# Autodesk Inventor assembly: 110202 DT-20-L1260ZZ
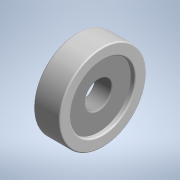
[picture p0: Inventor's stored thumbnail of the model, 180x180]
Saved by Autodesk Inventor 2022.3 (Build 263350000, 350)
## iProperties
Category: PARTsolutions
Company: TOKBEARING
Part Number: 110202 DT-20-L1260ZZ
Catalog Web Link: www.cadenas.de
Description: DT-
Vendor: TOKBEARING
Document SubType Name: Assembly
Designer: partserver
Manufacturer: TOKBEARING
Mass: 1.42292 g
Surface Area: 16.3578 cm^2
Volume: 1.42292 cm^3
Density: 1 g/cm^3
PSOL_IDENT_0: {$CADENAS_DATA\23d-libs\tok_bearing\i_series_bearings\dt_asmtab.prj},192 {VTYP=3D},{STYP=ASSTAB},{NB=
PSOL_IDENT_1: 110202 DT-20-L1260ZZ},{LINA=110202 DT-20-L1260ZZ},{NN=DT},{DATE=16.12.2020 00:38:07},{GEOMDATE=29.07
PSOL_IDENT_2: .2014 09:57:49},{VERSION=},{LINEID=2930},{WBVAR=},{WBNUMERIC=}  {NB=110202 DT-20-L1260ZZ},{LINA=1102
PSOL_IDENT_3: 02 DT-20-L1260ZZ},{KT=DUMMY},{IDNR=},{CODE=110202},{PN=DT-20-L1260ZZ},{D=20},{SD=6},{SDX=6.000},{W=6
PSOL_IDENT_4: },{C=-},{CX=0.000},{L=-},{LX=0.000},{N=-},{NX=0.000},{TYPE=1},{B=4},{BD=4},{OP=35.168},{BQ=5},{R=5.6
PSOL_IDENT_5: },{GP=2.4},{PPATH=dt/dt_asmtpl.prj}
NB: 110202 DT-20-L1260ZZ
NN: DT
NBSYN: $CODE. $PN.
LINA: 110202 DT-20-L1260ZZ
CATALOG: TOK, Inc
CODE: 110202
PN: DT-20-L1260ZZ
D: 20
SD: 6
W: 6
C: -
L: -
N: -
TYPE: 1
B: 4
SUPPLIER: TOKBEARING
ARTICLENO: 110202 DT-20-L1260ZZ
BOMINFO: 110202 DT-20-L1260ZZ
CREATOR: CADENAS GmbH
Title: 110202 DT-20-L1260ZZ
Author: Cadenas PARTsolutions
## Documents named in this file (3)
- C:\Users\YusukeKunita\Documents\GrabCAD\Development\BasicParts\Bearing\DT-20-L1260ZZ\DT-20-L1260ZZ.iam
- C:\Users\YusukeKunita\Documents\GrabCAD\Development\BasicParts\Bearing\DT-20-L1260ZZ\DT-20-L1260ZZ_or.ipt
- C:\Users\YusukeKunita\Documents\GrabCAD\Development\BasicParts\Bearing\DT-20-L1260ZZ\DT-20-L1260ZZ_ball.ipt
## Components (2 placed, 2 different names)
1. DT-20-L1260ZZ_or:1 — IP_roller_typ1_XY@1 <-> IP_ball_XY@2, IP_roller_typ1_Z@1 <-> IP_ball_Z@2, IP_roller_typ1_YZ@1 <-> IP_ball_YZ@2
2. DT-20-L1260ZZ_ball:1 — IP_roller_typ1_XY@1 <-> IP_ball_XY@2, IP_roller_typ1_Z@1 <-> IP_ball_Z@2, IP_roller_typ1_YZ@1 <-> IP_ball_YZ@2
## Relationships (3: Mate 2, Angle 1)
- IP_roller_typ1_XY@1 <-> IP_ball_XY@2 [Mate]: DT-20-L1260ZZ_or:1 ↔ DT-20-L1260ZZ_ball:1
- IP_roller_typ1_Z@1 <-> IP_ball_Z@2 [Mate]: DT-20-L1260ZZ_or:1 ↔ DT-20-L1260ZZ_ball:1
- IP_roller_typ1_YZ@1 <-> IP_ball_YZ@2 [Angle] (0 deg): DT-20-L1260ZZ_or:1 ↔ DT-20-L1260ZZ_ball:1
